# Autodesk Inventor assembly: fuse assem
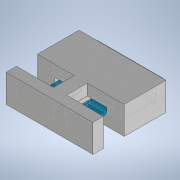
[picture p0: Inventor's stored thumbnail of the model, 180x180]
Saved by Autodesk Inventor 2021.5 (Build 255421000, 421)
## iProperties
Created: 2025-01-02
Part Number: fuse assem
Document SubType Name: Assembly
Designer: email
Author: email
## Documents named in this file (3)
- C:\Users\email\Desktop\Projects\Capstone\electornicsbox\fuse\fuse assem.iam
- C:\Users\email\Desktop\Projects\Capstone\electornicsbox\fusebox.ipt
- C:\Users\email\Desktop\Projects\Capstone\electornicsbox\fuse.ipt
## Components (2 placed, 2 different names)
1. fusebox:1 — Mate:1
2. fuse:1 — Mate:1
## Relationships (1: Mate 1)
- Mate:1: fusebox:1 ↔ fuse:1
